# Autodesk Inventor assembly: Placed 90 deg corner cabinet
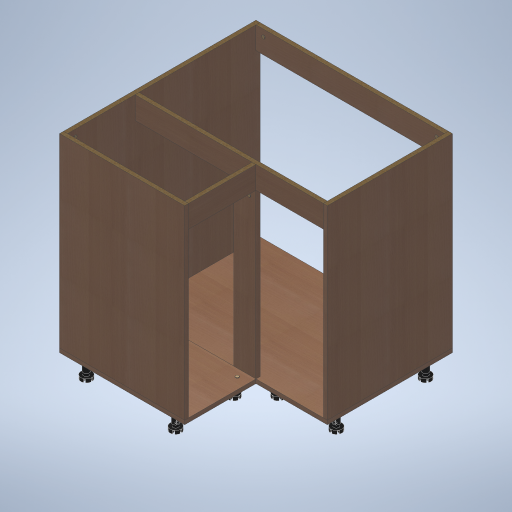
[picture p0: Inventor's stored thumbnail of the model, 512x512]
Saved by Autodesk Inventor 2024 (Build 280153000, 153)
## iProperties
RuleStatus: InUse
Created: 2017-01-30
Part Number: Placed 90 deg corner cabinet
Document SubType Name: Assembly
Designer: SvetlanaB
Author: SvetlanaB
## Documents named in this file (20)
- C:\W4INV 2024 Design\iBOX LIBRARY\Kitchen\Standing Cabinets\90 deg corner cabinet\Corner Cabinet.iam
- C:\W4INV 2024 Design\iBOX LIBRARY\Kitchen\Standing Cabinets\90 deg corner cabinet\Right panel.ipt
- C:\W4INV 2024 Design\iBOX LIBRARY\Kitchen\Standing Cabinets\90 deg corner cabinet\Left panel.ipt
- C:\W4INV 2024 Design\iBOX LIBRARY\Kitchen\Standing Cabinets\90 deg corner cabinet\Back panel_1.ipt
- C:\W4INV 2024 Design\iBOX LIBRARY\Kitchen\Standing Cabinets\90 deg corner cabinet\panel_1.ipt
- C:\W4INV 2024 Design\iBOX LIBRARY\Kitchen\Standing Cabinets\90 deg corner cabinet\Panel_2.ipt
- C:\W4INV 2024 Design\iBOX LIBRARY\Kitchen\Standing Cabinets\90 deg corner cabinet\Panel_3.ipt
- C:\W4INV 2024 Design\_LIBRARY\Fixed joints\Minifix joint\MINIFIX D15 v2\Minifix D15 & Dowel L34 & Cap D15 PB T18 LH.ipt
- C:\W4INV 2024 Design\_LIBRARY\Supports and legs\Legs\ADJUSTABLE LEG\Adjustable leg  BT18 clip included.ipt
- C:\W4INV 2024 Design\iBOX LIBRARY\Kitchen\Standing Cabinets\90 deg corner cabinet\Panel_4.ipt
- C:\W4INV 2024 Design\_LIBRARY\Fixed joints\Minifix joint\MINIFIX D15 v2\Minifix D15 & Dowel L34 & Cap D15 PB T18 RH.ipt
- C:\W4INV 2024 Design\_LIBRARY\Supports and legs\Legs\ADJUSTABLE LEG\Adjustable leg  BT18.ipt
- C:\W4INV 2024 Design\iBOX LIBRARY\Kitchen\Standing Cabinets\90 deg corner cabinet\corner cabinet concept.ipt
- C:\W4INV 2024 Design\iBOX LIBRARY\Kitchen\Standing Cabinets\90 deg corner cabinet\Bottom Panel 1.ipt
- C:\W4INV 2024 Design\iBOX LIBRARY\Kitchen\Standing Cabinets\90 deg corner cabinet\Bottom Panel 2.ipt
- C:\W4INV 2024 Design\_LIBRARY\Fixed joints\Confirmat\CONFIRMAT\Confirmat L50 & Cap D10 NB T18 PB T 18.ipt
- C:\W4INV 2024 Design\_LIBRARY\Fixed joints\Minifix joint\MINIFIX D15 v2\Minifix D15 & Dowel L34 & Cap D15 PB T18 BT.ipt
- C:\W4INV 2023 Design\LIBRARY\Fixed joints\Minifix joint\MINIFIX D15 v2.ipt
- C:\W4INV 2023 Design\LIBRARY\Fixed joints\Confirmat\CONFIRMAT.ipt
- C:\W4INV 2023 Design\LIBRARY\Supports and legs\Legs\ADJUSTABLE LEG.ipt
## Components (40 placed, 16 different names)
1. @Skeleton
2. Right panel:1 — Flush:4, Flush:29, Nestled Board Plane:9, Nestled Board Plane:12, Pillar Board Side Plane:4, Pillar Board Side Plane:6
3. Left panel:1 — Flush:2, Flush:27, Nestled Board Plane:7, Pillar Board Side Plane:7, Pillar Board Side Plane:8, Nestled Board Plane:17
4. Back panel_1:1 — Flush:10, Flush:11, Nestled Board Plane:11, Nestled Board Plane:14, Pillar Board Side Plane:3, Pillar Board Side Plane:5, Pillar Board Side Plane :1, Pillar Board Side Plane:11, Pillar Board Side Plane:12
5. panel_1:1 — Flush:5, Pillar Board Side Plane :9, Pillar Board Side Plane :10
6. Panel_2:1 — Pillar Board Side Plane :11, Pillar Board Side Plane :12, Nestled Board Plane:1, Nestled Board Plane:2, Nestled Board Plane:3
7. Panel_3:1 — Flush:54, Pillar Board Side Plane :7, Flush:65, Pillar Board Side Plane:1, Pillar Board Side Plane:2
8. Panel_4:1 — Flush:43, Flush:57, Flush:68, Pillar Board Side Plane :8, Pillar Board Side Plane:9, Pillar Board Side Plane:10
9. Minifix D15 & Dowel L34 & Cap D15 PB T18 LH:16 — Axis Plane:7, Nestled Board Plane:7, Pillar Board Side Plane :7
10. Minifix D15 & Dowel L34 & Cap D15 PB T18 LH:18 — Axis Plane:9, Nestled Board Plane:9, Pillar Board Side Plane :9
11. Minifix D15 & Dowel L34 & Cap D15 PB T18 RH:19 — Axis Plane:11, Nestled Board Plane:11, Pillar Board Side Plane :10
12. Minifix D15 & Dowel L34 & Cap D15 PB T18 RH:20 — Nestled Board Plane:12, Pillar Board Side Plane :11, Axis Plane:12
13. Minifix D15 & Dowel L34 & Cap D15 PB T18 LH:21 — Nestled Board Plane:14, Pillar Board Side Plane :12, Axis Plane:20
14. Bottom Panel 1:1 — Flush:66, Flush:67, Pillar Board Side Plane :14, Pillar Board Side Plane :15, Flush:78, Flush:79, Flush:80, Nestled Board Plane:15, Nestled Board Plane:16, Bottom board Plane:5, Front (Angle) Plane:5, Bottom board Plane:6, Front (Angle) Plane:6, Bottom board Plane:7, Front (Angle) Plane:7, Bottom board Plane:8, Front (Angle) Plane:8, Axis2 Plane:9, Pillar Board Side Plane :2, Flush:93, Nestled Board Plane:21, Nestled Board Plane:22
15. Bottom Panel 2:1 — Nestled Board Plane:4, Nestled Board Plane:5, Flush:76, Flush:77, Flush:81, Flush:82, Nestled Board Plane:6, Nestled Board Plane:8, Nestled Board Plane:10, Nestled Board Plane:13, Bottom board Plane:1, Front (Angle) Plane:1, Bottom board Plane:3, Front (Angle) Plane:3, Bottom board Plane:4, Front (Angle) Plane:4, Axis2 Plane:7, Axis2 Plane:8, Bottom board Plane:9, Front (Angle) Plane:9, Nestled Board Plane:18, Nestled Board Plane:19, Nestled Board Plane:20
16. Confirmat L50 & Cap D10 NB T18 PB T 18:1 — Axis Plane:8, Pillar Board Side Plane:1, Nestled Board Plane:1
17. Confirmat L50 & Cap D10 NB T18 PB T 18:2 — Axis Plane:21, Pillar Board Side Plane:2, Nestled Board Plane:2
18. Minifix D15 & Dowel L34 & Cap D15 PB T18 RH:23 — Nestled Board Plane:3, Pillar Board Side Plane :8, Axis Plane:22
19. Minifix D15 & Dowel L34 & Cap D15 PB T18 RH:24 — Nestled Board Plane:4, Pillar Board Side Plane :14, Axis Plane:23
20. Minifix D15 & Dowel L34 & Cap D15 PB T18 LH:25 — Axis Plane:24, Nestled Board Plane:5, Pillar Board Side Plane :15
21. Confirmat L50 & Cap D10 NB T18 PB T 18:3 — Axis Plane:1, Pillar Board Side Plane:3, Nestled Board Plane:6
22. Confirmat L50 & Cap D10 NB T18 PB T 18:4 — Axis Plane:2, Pillar Board Side Plane:4, Nestled Board Plane:8
23. Confirmat L50 & Cap D10 NB T18 PB T 18:5 — Axis Plane:3, Pillar Board Side Plane:5, Nestled Board Plane:10
24. Confirmat L50 & Cap D10 NB T18 PB T 18:6 — Axis Plane:4, Pillar Board Side Plane:6, Nestled Board Plane:13
25. Confirmat L50 & Cap D10 NB T18 PB T 18:7 — Axis Plane:5, Nestled Board Plane:15, Pillar Board Side Plane:7
26. Confirmat L50 & Cap D10 NB T18 PB T 18:8 — Axis Plane:6, Nestled Board Plane:16, Pillar Board Side Plane:8
27. Minifix D15 & Dowel L34 & Cap D15 PB T18 RH:26 — Nestled Board Plane:17, Pillar Board Side Plane :1, Axis Plane:13
28. Adjustable leg  BT18 clip included:1 — Axis2 Plane:1, Axis Plane:14, Bottom board Plane:1, Front (Angle) Plane:1
29. Adjustable leg  BT18:3 — Axis2 Plane:3, Axis Plane:16, Bottom board Plane:3, Front (Angle) Plane:3
30. Adjustable leg  BT18:4 — Axis2 Plane:4, Axis Plane:17, Bottom board Plane:4, Front (Angle) Plane:4
31. Adjustable leg  BT18:5 — Axis2 Plane:5, Bottom board Plane:5, Axis Plane:18, Front (Angle) Plane:5
32. Adjustable leg  BT18 clip included:6 — Axis2 Plane:6, Bottom board Plane:6, Axis Plane:19, Front (Angle) Plane:6
33. Adjustable leg  BT18 clip included:7 — Axis Plane:25, Bottom board Plane:7, Axis2 Plane:7, Front (Angle) Plane:7
34. Adjustable leg  BT18:8 — Axis Plane:26, Bottom board Plane:8, Axis2 Plane:8, Front (Angle) Plane:8
35. Adjustable leg  BT18 clip included:9 — Bottom board Plane:9, Axis Plane:27, Axis2 Plane:9, Front (Angle) Plane:9
36. Confirmat L50 & Cap D10 NB T18 PB T 18:10 — Axis Plane:10, Nestled Board Plane:18, Pillar Board Side Plane:9
37. Confirmat L50 & Cap D10 NB T18 PB T 18:11 — Axis Plane:28, Nestled Board Plane:19, Pillar Board Side Plane:10
38. Minifix D15 & Dowel L34 & Cap D15 PB T18 BT:27 — Nestled Board Plane:20, Pillar Board Side Plane :2, Axis Plane:29
39. Confirmat L50 & Cap D10 NB T18 PB T 18:12 — Axis Plane:30, Nestled Board Plane:21, Pillar Board Side Plane:11
40. Confirmat L50 & Cap D10 NB T18 PB T 18:13 — Axis Plane:31, Nestled Board Plane:22, Pillar Board Side Plane:12
## Relationships (122: Mate 68, Flush 44, Angle 8, Symmetry 2)
- Flush:2 (-64 mm): Left panel:1
- Flush:4 (-64 mm): Right panel:1
- Flush:5 (-30 mm): panel_1:1
- Flush:10 (-64 mm): Back panel_1:1
- Flush:11 (-64 mm): Back panel_1:1
- Flush:27 (-64 mm): Left panel:1
- Flush:29 (-64 mm): Right panel:1
- Flush:43 (-20 mm): Panel_4:1
- Flush:54 (-30 mm): Panel_3:1
- Flush:57 (-30 mm): Panel_4:1
- Axis Plane:7 [Mate]: Minifix D15 & Dowel L34 & Cap D15 PB T18 LH:16
- Nestled Board Plane:7 [Mate]: Left panel:1 ↔ Minifix D15 & Dowel L34 & Cap D15 PB T18 LH:16
- Pillar Board Side Plane :7 [Flush] (18 mm): Panel_3:1 ↔ Minifix D15 & Dowel L34 & Cap D15 PB T18 LH:16
- Axis Plane:9 [Mate]: Minifix D15 & Dowel L34 & Cap D15 PB T18 LH:18
- Nestled Board Plane:9 [Mate]: Right panel:1 ↔ Minifix D15 & Dowel L34 & Cap D15 PB T18 LH:18
- Pillar Board Side Plane :9 [Flush] (18 mm): panel_1:1 ↔ Minifix D15 & Dowel L34 & Cap D15 PB T18 LH:18
- Axis Plane:11 [Mate]: Minifix D15 & Dowel L34 & Cap D15 PB T18 RH:19
- Nestled Board Plane:11 [Mate]: Back panel_1:1 ↔ Minifix D15 & Dowel L34 & Cap D15 PB T18 RH:19
- Pillar Board Side Plane :10 [Flush] (18 mm): panel_1:1 ↔ Minifix D15 & Dowel L34 & Cap D15 PB T18 RH:19
- Nestled Board Plane:12 [Mate]: Right panel:1 ↔ Minifix D15 & Dowel L34 & Cap D15 PB T18 RH:20
- Pillar Board Side Plane :11 [Flush] (18 mm): Panel_2:1 ↔ Minifix D15 & Dowel L34 & Cap D15 PB T18 RH:20
- Axis Plane:12 [Mate]: Minifix D15 & Dowel L34 & Cap D15 PB T18 RH:20
- Nestled Board Plane:14 [Mate]: Back panel_1:1 ↔ Minifix D15 & Dowel L34 & Cap D15 PB T18 LH:21
- Pillar Board Side Plane :12 [Flush] (18 mm): Panel_2:1 ↔ Minifix D15 & Dowel L34 & Cap D15 PB T18 LH:21
- Axis Plane:20 [Mate]: Minifix D15 & Dowel L34 & Cap D15 PB T18 LH:21
- Flush:65 (-30 mm): Panel_3:1
- Flush:66 (-100 mm): Bottom Panel 1:1
- Flush:67 (-60 mm): Bottom Panel 1:1
- Flush:68 (-30 mm): Panel_4:1
- Axis Plane:8 [Mate]: Confirmat L50 & Cap D10 NB T18 PB T 18:1
- Pillar Board Side Plane:1 [Mate] (-9 mm): Panel_3:1 ↔ Confirmat L50 & Cap D10 NB T18 PB T 18:1
- Axis Plane:21 [Mate]: Confirmat L50 & Cap D10 NB T18 PB T 18:2
- Pillar Board Side Plane:2 [Mate] (-9 mm): Panel_3:1 ↔ Confirmat L50 & Cap D10 NB T18 PB T 18:2
- Nestled Board Plane:1 [Flush]: Panel_2:1 ↔ Confirmat L50 & Cap D10 NB T18 PB T 18:1
- Nestled Board Plane:2 [Flush]: Panel_2:1 ↔ Confirmat L50 & Cap D10 NB T18 PB T 18:2
- Nestled Board Plane:3 [Mate]: Panel_2:1 ↔ Minifix D15 & Dowel L34 & Cap D15 PB T18 RH:23
- Pillar Board Side Plane :8 [Flush] (18 mm): Panel_4:1 ↔ Minifix D15 & Dowel L34 & Cap D15 PB T18 RH:23
- Axis Plane:22 [Mate]: Minifix D15 & Dowel L34 & Cap D15 PB T18 RH:23
- Nestled Board Plane:4 [Mate]: Bottom Panel 2:1 ↔ Minifix D15 & Dowel L34 & Cap D15 PB T18 RH:24
- Pillar Board Side Plane :14 [Flush] (18 mm): Bottom Panel 1:1 ↔ Minifix D15 & Dowel L34 & Cap D15 PB T18 RH:24
- Axis Plane:24 [Mate]: Minifix D15 & Dowel L34 & Cap D15 PB T18 LH:25
- Nestled Board Plane:5 [Mate]: Bottom Panel 2:1 ↔ Minifix D15 & Dowel L34 & Cap D15 PB T18 LH:25
- Pillar Board Side Plane :15 [Flush] (18 mm): Bottom Panel 1:1 ↔ Minifix D15 & Dowel L34 & Cap D15 PB T18 LH:25
- Symmetry:1
- Axis Plane:23 [Mate]: Minifix D15 & Dowel L34 & Cap D15 PB T18 RH:24
- Flush:76 (-100 mm): Bottom Panel 2:1
- Flush:77 (-60 mm): Bottom Panel 2:1
- Flush:78 (-100 mm): Bottom Panel 1:1
- Flush:79 (-60 mm): Bottom Panel 1:1
- Flush:80 (-60 mm): Bottom Panel 1:1
- Flush:81 (-60 mm): Bottom Panel 2:1
- Flush:82 (-60 mm): Bottom Panel 2:1
- Axis Plane:1 [Mate]: Confirmat L50 & Cap D10 NB T18 PB T 18:3
- Pillar Board Side Plane:3 [Mate] (-9 mm): Back panel_1:1 ↔ Confirmat L50 & Cap D10 NB T18 PB T 18:3
- Nestled Board Plane:6 [Flush]: Bottom Panel 2:1 ↔ Confirmat L50 & Cap D10 NB T18 PB T 18:3
- Axis Plane:2 [Mate]: Confirmat L50 & Cap D10 NB T18 PB T 18:4
- Pillar Board Side Plane:4 [Mate] (-9 mm): Right panel:1 ↔ Confirmat L50 & Cap D10 NB T18 PB T 18:4
- Nestled Board Plane:8 [Flush]: Bottom Panel 2:1 ↔ Confirmat L50 & Cap D10 NB T18 PB T 18:4
- Axis Plane:3 [Mate]: Confirmat L50 & Cap D10 NB T18 PB T 18:5
- Pillar Board Side Plane:5 [Mate] (-9 mm): Back panel_1:1 ↔ Confirmat L50 & Cap D10 NB T18 PB T 18:5
- Nestled Board Plane:10 [Flush]: Bottom Panel 2:1 ↔ Confirmat L50 & Cap D10 NB T18 PB T 18:5
- Axis Plane:4 [Mate]: Confirmat L50 & Cap D10 NB T18 PB T 18:6
- Pillar Board Side Plane:6 [Mate] (-9 mm): Right panel:1 ↔ Confirmat L50 & Cap D10 NB T18 PB T 18:6
- Nestled Board Plane:13 [Flush]: Bottom Panel 2:1 ↔ Confirmat L50 & Cap D10 NB T18 PB T 18:6
- Axis Plane:5 [Mate]: Confirmat L50 & Cap D10 NB T18 PB T 18:7
- Nestled Board Plane:15 [Flush]: Bottom Panel 1:1 ↔ Confirmat L50 & Cap D10 NB T18 PB T 18:7
- Pillar Board Side Plane:7 [Mate] (-9 mm): Left panel:1 ↔ Confirmat L50 & Cap D10 NB T18 PB T 18:7
- Axis Plane:6 [Mate]: Confirmat L50 & Cap D10 NB T18 PB T 18:8
- Nestled Board Plane:16 [Flush]: Bottom Panel 1:1 ↔ Confirmat L50 & Cap D10 NB T18 PB T 18:8
- Pillar Board Side Plane:8 [Mate] (-9 mm): Left panel:1 ↔ Confirmat L50 & Cap D10 NB T18 PB T 18:8
- Nestled Board Plane:17 [Mate]: Left panel:1 ↔ Minifix D15 & Dowel L34 & Cap D15 PB T18 RH:26
- Pillar Board Side Plane :1 [Flush] (18 mm): Back panel_1:1 ↔ Minifix D15 & Dowel L34 & Cap D15 PB T18 RH:26
- Axis Plane:13 [Mate]: Minifix D15 & Dowel L34 & Cap D15 PB T18 RH:26
- Axis2 Plane:1 [Mate]: Adjustable leg  BT18 clip included:1
- Axis Plane:14 [Mate]: Adjustable leg  BT18 clip included:1
- Bottom board Plane:1 [Mate]: Bottom Panel 2:1 ↔ Adjustable leg  BT18 clip included:1
- Front (Angle) Plane:1 [Angle] (0 deg): Bottom Panel 2:1 ↔ Adjustable leg  BT18 clip included:1
- Axis2 Plane:3 [Mate]: Adjustable leg  BT18:3
- Axis Plane:16 [Mate]: Adjustable leg  BT18:3
- Bottom board Plane:3 [Mate]: Bottom Panel 2:1 ↔ Adjustable leg  BT18:3
- Front (Angle) Plane:3 [Angle] (0 deg): Bottom Panel 2:1 ↔ Adjustable leg  BT18:3
- Axis2 Plane:4 [Mate]: Adjustable leg  BT18:4
- Axis Plane:17 [Mate]: Adjustable leg  BT18:4
- Bottom board Plane:4 [Mate]: Bottom Panel 2:1 ↔ Adjustable leg  BT18:4
- Front (Angle) Plane:4 [Angle] (0 deg): Bottom Panel 2:1 ↔ Adjustable leg  BT18:4
- Axis2 Plane:5 [Mate]: Adjustable leg  BT18:5
- Bottom board Plane:5 [Mate]: Bottom Panel 1:1 ↔ Adjustable leg  BT18:5
- Axis Plane:18 [Mate]: Adjustable leg  BT18:5
- Front (Angle) Plane:5 [Angle] (0 deg): Bottom Panel 1:1 ↔ Adjustable leg  BT18:5
- Axis2 Plane:6 [Mate]: Adjustable leg  BT18 clip included:6
- Bottom board Plane:6 [Mate]: Bottom Panel 1:1 ↔ Adjustable leg  BT18 clip included:6
- Axis Plane:19 [Mate]: Adjustable leg  BT18 clip included:6
- Front (Angle) Plane:6 [Angle] (0 deg): Bottom Panel 1:1 ↔ Adjustable leg  BT18 clip included:6
- Axis Plane:25 [Mate]: Adjustable leg  BT18 clip included:7
- Bottom board Plane:7 [Mate]: Bottom Panel 1:1 ↔ Adjustable leg  BT18 clip included:7
- Axis2 Plane:7 [Mate]: Bottom Panel 2:1 ↔ Adjustable leg  BT18 clip included:7
- Front (Angle) Plane:7 [Angle] (0 deg): Bottom Panel 1:1 ↔ Adjustable leg  BT18 clip included:7
- Axis Plane:26 [Mate]: Adjustable leg  BT18:8
- Bottom board Plane:8 [Mate]: Bottom Panel 1:1 ↔ Adjustable leg  BT18:8
- Axis2 Plane:8 [Mate]: Bottom Panel 2:1 ↔ Adjustable leg  BT18:8
- Front (Angle) Plane:8 [Angle] (0 deg): Bottom Panel 1:1 ↔ Adjustable leg  BT18:8
- Bottom board Plane:9 [Mate]: Bottom Panel 2:1 ↔ Adjustable leg  BT18 clip included:9
- Axis Plane:27 [Mate]: Adjustable leg  BT18 clip included:9
- Axis2 Plane:9 [Mate]: Bottom Panel 1:1 ↔ Adjustable leg  BT18 clip included:9
- Front (Angle) Plane:9 [Angle] (0 deg): Bottom Panel 2:1 ↔ Adjustable leg  BT18 clip included:9
- Axis Plane:10 [Mate]: Confirmat L50 & Cap D10 NB T18 PB T 18:10
- Nestled Board Plane:18 [Flush]: Bottom Panel 2:1 ↔ Confirmat L50 & Cap D10 NB T18 PB T 18:10
- Pillar Board Side Plane:9 [Mate] (-9 mm): Panel_4:1 ↔ Confirmat L50 & Cap D10 NB T18 PB T 18:10
- Axis Plane:28 [Mate]: Confirmat L50 & Cap D10 NB T18 PB T 18:11
- Nestled Board Plane:19 [Flush]: Bottom Panel 2:1 ↔ Confirmat L50 & Cap D10 NB T18 PB T 18:11
- Pillar Board Side Plane:10 [Mate] (-9 mm): Panel_4:1 ↔ Confirmat L50 & Cap D10 NB T18 PB T 18:11
- Symmetry:2
- Nestled Board Plane:20 [Mate]: Bottom Panel 2:1 ↔ Minifix D15 & Dowel L34 & Cap D15 PB T18 BT:27
- Pillar Board Side Plane :2 [Flush] (18 mm): Bottom Panel 1:1 ↔ Minifix D15 & Dowel L34 & Cap D15 PB T18 BT:27
- Axis Plane:29 [Mate]: Minifix D15 & Dowel L34 & Cap D15 PB T18 BT:27
- Flush:93 (-60 mm): Bottom Panel 1:1
- Axis Plane:30 [Mate]: Confirmat L50 & Cap D10 NB T18 PB T 18:12
- Nestled Board Plane:21 [Flush]: Bottom Panel 1:1 ↔ Confirmat L50 & Cap D10 NB T18 PB T 18:12
- Pillar Board Side Plane:11 [Mate] (-9 mm): Back panel_1:1 ↔ Confirmat L50 & Cap D10 NB T18 PB T 18:12
- Axis Plane:31 [Mate]: Confirmat L50 & Cap D10 NB T18 PB T 18:13
- Nestled Board Plane:22 [Flush]: Bottom Panel 1:1 ↔ Confirmat L50 & Cap D10 NB T18 PB T 18:13
- Pillar Board Side Plane:12 [Mate] (-9 mm): Back panel_1:1 ↔ Confirmat L50 & Cap D10 NB T18 PB T 18:13
## Named parameters: Panel_thickness = 18 mm, Right_cupboard_side = 560 mm, Left_cupboard_side = 560 mm
